# Autodesk Inventor assembly: 0008-10-01 Sckeleton
(part 2 of 2)
- Insert:179: 0008-10-2012 DIN 125 - A 5.3.ipt:190 ↔ 0008-10-2013 DIN 7984 - M5 x 20.ipt:191
- Insert:180: 0008-10-035.ipt:27 ↔ 0008-10-2012 DIN 125 - A 5.3.ipt:190
- [Insert] (-5 mm): 0008-10-2010 M 5 Canal.ipt:192 ↔ 0008-10-2013 DIN 7984 - M5 x 20.ipt:194
- [Insert]: 0008-10-2012 DIN 125 - A 5.3.ipt:193 ↔ 0008-10-2013 DIN 7984 - M5 x 20.ipt:194
- Mate:182: 0008-10-035.ipt:27 ↔ 0008-10-2012 DIN 125 - A 5.3.ipt:193
- [Insert] (-5 mm): 0008-10-2010 M 5 Canal.ipt:195 ↔ 0008-10-2013 DIN 7984 - M5 x 20.ipt:197
- [Insert]: 0008-10-2012 DIN 125 - A 5.3.ipt:196 ↔ 0008-10-2013 DIN 7984 - M5 x 20.ipt:197
- [Insert] (-5 mm): 0008-10-2010 M 5 Canal.ipt:198 ↔ 0008-10-2013 DIN 7984 - M5 x 20.ipt:200
- [Insert]: 0008-10-2012 DIN 125 - A 5.3.ipt:199 ↔ 0008-10-2013 DIN 7984 - M5 x 20.ipt:200
- Insert:187: 0008-10-035.ipt:27 ↔ 0008-10-2012 DIN 125 - A 5.3.ipt:199
- Insert:188: 0008-10-035.ipt:27 ↔ 0008-10-2012 DIN 125 - A 5.3.ipt:196
- [Insert] (-5 mm): 0008-10-2010 M 5 Canal.ipt:201 ↔ 0008-10-2013 DIN 7984 - M5 x 20.ipt:203
- [Insert]: 0008-10-2012 DIN 125 - A 5.3.ipt:202 ↔ 0008-10-2013 DIN 7984 - M5 x 20.ipt:203
- [Insert] (-5 mm): 0008-10-2010 M 5 Canal.ipt:204 ↔ 0008-10-2013 DIN 7984 - M5 x 20.ipt:206
- [Insert]: 0008-10-2012 DIN 125 - A 5.3.ipt:205 ↔ 0008-10-2013 DIN 7984 - M5 x 20.ipt:206
- [Insert] (-5 mm): 0008-10-2010 M 5 Canal.ipt:207 ↔ 0008-10-2013 DIN 7984 - M5 x 20.ipt:209
- [Insert]: 0008-10-2012 DIN 125 - A 5.3.ipt:208 ↔ 0008-10-2013 DIN 7984 - M5 x 20.ipt:209
- [Insert] (-5 mm): 0008-10-2010 M 5 Canal.ipt:210 ↔ 0008-10-2013 DIN 7984 - M5 x 20.ipt:212
- [Insert]: 0008-10-2012 DIN 125 - A 5.3.ipt:211 ↔ 0008-10-2013 DIN 7984 - M5 x 20.ipt:212
- Insert:197: 0008-10-033.ipt:26 ↔ 0008-10-2012 DIN 125 - A 5.3.ipt:211
- Insert:198: 0008-10-033.ipt:26 ↔ 0008-10-2012 DIN 125 - A 5.3.ipt:202
- Insert:199: 0008-10-033.ipt:26 ↔ 0008-10-2012 DIN 125 - A 5.3.ipt:208
- Insert:200: 0008-10-033.ipt:26 ↔ 0008-10-2012 DIN 125 - A 5.3.ipt:205
- Insert:224: 0008-10-024 Ranforsare.ipt:16 ↔ 0008-10-2012 DIN 125 - A 5.3.ipt:218
- Insert:225: 0008-10-2012 DIN 125 - A 5.3.ipt:218 ↔ 0008-10-2014 DIN 7984 - M5 x 25.ipt:222
- [Insert]: 0008-10-2012 DIN 125 - A 5.3.ipt:223 ↔ 0008-10-2014 DIN 7984 - M5 x 25.ipt:224
- Insert:227: 0008-10-024 Ranforsare.ipt:16 ↔ 0008-10-2012 DIN 125 - A 5.3.ipt:223
- [Insert]: 0008-10-2012 DIN 125 - A 5.3.ipt:225 ↔ 0008-10-2014 DIN 7984 - M5 x 25.ipt:226
- [Insert]: 0008-10-2012 DIN 125 - A 5.3.ipt:227 ↔ 0008-10-2014 DIN 7984 - M5 x 25.ipt:228
- Insert:230: 0008-10-024 Ranforsare.ipt:18 ↔ 0008-10-2012 DIN 125 - A 5.3.ipt:227
- Insert:231: 0008-10-024 Ranforsare.ipt:18 ↔ 0008-10-2012 DIN 125 - A 5.3.ipt:225
- [Insert]: 0008-10-2012 DIN 125 - A 5.3.ipt:229 ↔ 0008-10-2014 DIN 7984 - M5 x 25.ipt:230
- [Insert]: 0008-10-2012 DIN 125 - A 5.3.ipt:231 ↔ 0008-10-2014 DIN 7984 - M5 x 25.ipt:232
- [Insert]: 0008-10-2012 DIN 125 - A 5.3.ipt:233 ↔ 0008-10-2014 DIN 7984 - M5 x 25.ipt:234
- Insert:235: 0008-10-024 Ranforsare.ipt:15 ↔ 0008-10-2012 DIN 125 - A 5.3.ipt:233
- Insert:236: 0008-10-024 Ranforsare.ipt:15 ↔ 0008-10-2012 DIN 125 - A 5.3.ipt:231
- Insert:237: 0008-10-024 Ranforsare.ipt:17 ↔ 0008-10-2012 DIN 125 - A 5.3.ipt:229
- [Insert]: 0008-10-2012 DIN 125 - A 5.3.ipt:235 ↔ 0008-10-2014 DIN 7984 - M5 x 25.ipt:236
- Insert:239: 0008-10-024 Ranforsare.ipt:17 ↔ 0008-10-2012 DIN 125 - A 5.3.ipt:235
- Insert:240 (-2 mm): 0008-10-2010 M 5 Canal.ipt:237 ↔ 0008-10-2015 DIN 7984 - M5 x 8.ipt:239
- Insert:241: 0008-10-2012 DIN 125 - A 5.3.ipt:238 ↔ 0008-10-2015 DIN 7984 - M5 x 8.ipt:239
- Insert:242: 0008-10-022 Tabla suport.ipt:10 ↔ 0008-10-2012 DIN 125 - A 5.3.ipt:238
- [Insert] (-2 mm): 0008-10-2010 M 5 Canal.ipt:240 ↔ 0008-10-2015 DIN 7984 - M5 x 8.ipt:242
- [Insert]: 0008-10-2012 DIN 125 - A 5.3.ipt:241 ↔ 0008-10-2015 DIN 7984 - M5 x 8.ipt:242
- [Insert] (-2 mm): 0008-10-2010 M 5 Canal.ipt:243 ↔ 0008-10-2015 DIN 7984 - M5 x 8.ipt:245
- [Insert]: 0008-10-2012 DIN 125 - A 5.3.ipt:244 ↔ 0008-10-2015 DIN 7984 - M5 x 8.ipt:245
- [Insert] (-2 mm): 0008-10-2010 M 5 Canal.ipt:246 ↔ 0008-10-2015 DIN 7984 - M5 x 8.ipt:248
- [Insert]: 0008-10-2012 DIN 125 - A 5.3.ipt:247 ↔ 0008-10-2015 DIN 7984 - M5 x 8.ipt:248
- [Insert] (-2 mm): 0008-10-2010 M 5 Canal.ipt:249 ↔ 0008-10-2015 DIN 7984 - M5 x 8.ipt:251
- [Insert]: 0008-10-2012 DIN 125 - A 5.3.ipt:250 ↔ 0008-10-2015 DIN 7984 - M5 x 8.ipt:251
- [Insert] (-2 mm): 0008-10-2010 M 5 Canal.ipt:252 ↔ 0008-10-2015 DIN 7984 - M5 x 8.ipt:254
- [Insert]: 0008-10-2012 DIN 125 - A 5.3.ipt:253 ↔ 0008-10-2015 DIN 7984 - M5 x 8.ipt:254
- [Insert] (-2 mm): 0008-10-2010 M 5 Canal.ipt:255 ↔ 0008-10-2015 DIN 7984 - M5 x 8.ipt:257
- [Insert]: 0008-10-2012 DIN 125 - A 5.3.ipt:256 ↔ 0008-10-2015 DIN 7984 - M5 x 8.ipt:257
- [Insert] (-2 mm): 0008-10-2010 M 5 Canal.ipt:258 ↔ 0008-10-2015 DIN 7984 - M5 x 8.ipt:260
- [Insert]: 0008-10-2012 DIN 125 - A 5.3.ipt:259 ↔ 0008-10-2015 DIN 7984 - M5 x 8.ipt:260
- [Insert] (-2 mm): 0008-10-2010 M 5 Canal.ipt:261 ↔ 0008-10-2015 DIN 7984 - M5 x 8.ipt:263
- [Insert]: 0008-10-2012 DIN 125 - A 5.3.ipt:262 ↔ 0008-10-2015 DIN 7984 - M5 x 8.ipt:263
- [Insert] (-2 mm): 0008-10-2010 M 5 Canal.ipt:264 ↔ 0008-10-2015 DIN 7984 - M5 x 8.ipt:266
- [Insert]: 0008-10-2012 DIN 125 - A 5.3.ipt:265 ↔ 0008-10-2015 DIN 7984 - M5 x 8.ipt:266
- [Insert] (-2 mm): 0008-10-2010 M 5 Canal.ipt:267 ↔ 0008-10-2015 DIN 7984 - M5 x 8.ipt:269
- [Insert]: 0008-10-2012 DIN 125 - A 5.3.ipt:268 ↔ 0008-10-2015 DIN 7984 - M5 x 8.ipt:269
- [Insert] (-2 mm): 0008-10-2010 M 5 Canal.ipt:270 ↔ 0008-10-2015 DIN 7984 - M5 x 8.ipt:272
- [Insert]: 0008-10-2012 DIN 125 - A 5.3.ipt:271 ↔ 0008-10-2015 DIN 7984 - M5 x 8.ipt:272
- Insert:265: 0008-10-022 Tabla suport.ipt:10 ↔ 0008-10-2012 DIN 125 - A 5.3.ipt:241
- Insert:266: 0008-10-022 Tabla suport.ipt:10 ↔ 0008-10-2012 DIN 125 - A 5.3.ipt:244
- Insert:267: 0008-10-022 Tabla suport.ipt:10 ↔ 0008-10-2012 DIN 125 - A 5.3.ipt:247
- Insert:268: 0008-10-022 Tabla suport.ipt:10 ↔ 0008-10-2012 DIN 125 - A 5.3.ipt:250
- Insert:269: 0008-10-022 Tabla suport.ipt:10 ↔ 0008-10-2012 DIN 125 - A 5.3.ipt:253
- Insert:270: 0008-10-022 Tabla suport.ipt:10 ↔ 0008-10-2012 DIN 125 - A 5.3.ipt:256
- Insert:271: 0008-10-022 Tabla suport.ipt:10 ↔ 0008-10-2012 DIN 125 - A 5.3.ipt:268
- Insert:272: 0008-10-022 Tabla suport.ipt:10 ↔ 0008-10-2012 DIN 125 - A 5.3.ipt:259
- Insert:273: 0008-10-022 Tabla suport.ipt:10 ↔ 0008-10-2012 DIN 125 - A 5.3.ipt:262
- Insert:274: 0008-10-022 Tabla suport.ipt:10 ↔ 0008-10-2012 DIN 125 - A 5.3.ipt:265
- Insert:275: 0008-10-022 Tabla suport.ipt:10 ↔ 0008-10-2012 DIN 125 - A 5.3.ipt:271
## Named parameters: d458_d455 = -5 mm, d459_d456 = 0 mm, d460_d455 = -5 mm, d461_d456 = 0 mm, d462_d455 = -5 mm, d463_d456 = 0 mm, d464_d455 = -5 mm, d465_d456 = 0 mm, d470_d455 = -5 mm, d471_d456 = 0 mm, d472_d455 = -5 mm, d473_d456 = 0 mm, d474_d455 = -5 mm, d475_d456 = 0 mm, d479_d455 = -5 mm, d480_d456 = 0 mm, d481_d455 = -5 mm, d482_d456 = 0 mm, d483_d455 = -5 mm, d484_d456 = 0 mm, d485_d455 = -5 mm, d486_d456 = 0 mm, d491_d455 = -5 mm, d492_d456 = 0 mm, d493_d455 = -5 mm, d494_d456 = 0 mm, d495_d455 = -5 mm, d496_d456 = 0 mm, d497_d455 = -5 mm, d498_d456 = 0 mm, d503_d455 = -5 mm, d504_d456 = 0 mm, d505_d455 = -5 mm, d506_d456 = 0 mm, d507_d455 = -5 mm, d508_d456 = 0 mm, d509_d455 = -5 mm, d510_d456 = 0 mm, d511_d455 = -5 mm, d512_d456 = 0 mm, d513_d455 = -5 mm, d514_d456 = 0 mm, d515_d455 = -5 mm, d516_d456 = 0 mm, d517_d455 = -5 mm, d518_d456 = 0 mm, d519_d455 = -5 mm, d520_d456 = 0 mm, d521_d455 = -5 mm, d522_d456 = 0 mm, d523_d455 = -5 mm, d524_d456 = 0 mm, d525_d455 = -5 mm, d526_d456 = 0 mm, d539_d455 = -5 mm, d540_d456 = 0 mm, d541_d455 = -5 mm, d542_d456 = 0 mm, d543_d455 = -5 mm, d544_d456 = 0 mm, d545_d455 = -5 mm, d546_d456 = 0 mm, d551_d455 = -5 mm, d552_d456 = 0 mm, d553_d455 = -5 mm, d554_d456 = 0 mm, d555_d455 = -5 mm, d556_d456 = 0 mm, d557_d455 = -5 mm, d558_d456 = 0 mm, d559_d455 = -5 mm, d560_d456 = 0 mm, d561_d455 = -5 mm, d562_d456 = 0 mm, d563_d455 = -5 mm, d564_d456 = 0 mm, d565_d455 = -5 mm, d566_d456 = 0 mm, d567_d455 = -5 mm, d568_d456 = 0 mm, d569_d455 = -5 mm, d570_d456 = 0 mm, d571_d455 = -5 mm, d572_d456 = 0 mm, d573_d455 = -5 mm, d574_d456 = 0 mm, d587_d455 = -5 mm, d588_d456 = 0 mm, d589_d455 = -5 mm, d590_d456 = 0 mm, d591_d455 = -5 mm, d592_d456 = 0 mm, d593_d455 = -5 mm, d594_d456 = 0 mm, d602_d455 = -5 mm, d603_d456 = 0 mm, d604_d455 = -5 mm, d605_d456 = 0 mm, d606_d455 = -5 mm, d607_d456 = 0 mm, d608_d455 = -5 mm, d609_d456 = 0 mm, d619_d616 = -5 mm, d620_d617 = 0 mm, d622_d616 = -5 mm, d623_d617 = 0 mm, d624_d616 = -5 mm, d625_d617 = 0 mm, d628_d616 = -5 mm, d629_d617 = 0 mm, d630_d616 = -5 mm, d631_d617 = 0 mm, d632_d616 = -5 mm, d633_d617 = 0 mm, d634_d616 = -5 mm, d635_d617 = 0 mm, d667_d666 = 0 mm, d669_d666 = 0 mm, d670_d666 = 0 mm, d673_d666 = 0 mm, d674_d666 = 0 mm, d675_d666 = 0 mm, d679_d666 = 0 mm, d684_d681 = -2 mm, d685_d682 = 0 mm, d686_d681 = -2 mm, d687_d682 = 0 mm, d688_d681 = -2 mm, d689_d682 = 0 mm, d690_d681 = -2 mm, d691_d682 = 0 mm, d692_d681 = -2 mm, d693_d682 = 0 mm, d694_d681 = -2 mm, d695_d682 = 0 mm, d696_d681 = -2 mm, d697_d682 = 0 mm, d698_d681 = -2 mm, d699_d682 = 0 mm, d700_d681 = -2 mm, d701_d682 = 0 mm, d702_d681 = -2 mm, d703_d682 = 0 mm, d704_d681 = -2 mm, d705_d682 = 0 mm
